# Autodesk Inventor assembly: 276-2156
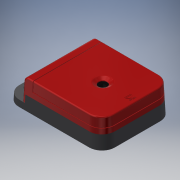
[picture p0: Inventor's stored thumbnail of the model, 180x180]
Saved by Autodesk Inventor 2019.4 (Build 234330000, 330)
## iProperties
Category: Sensors
Company: Autodesk Inc.
Created: 2012-04-02
Part Number: 276-2156
Document SubType Name: Assembly
Designer: Autodesk Inc.
Catalog Web Link: http://www.vexrobotics.com/276-2156.html
Vendor: VEX
Author: Autodesk Inc.
## Documents named in this file (7)
- D:\2019-2020TowerTakeOverCad\ncrCadLib\传感器\Optical Shaft Encoder.iam
- D:\2019-2020TowerTakeOverCad\ncrCadLib\传感器\Reference Parts\Shaft Encoder Bottom.ipt
- D:\2019-2020TowerTakeOverCad\ncrCadLib\传感器\Reference Parts\Optical Shaft Mid.ipt
- D:\2019-2020TowerTakeOverCad\ncrCadLib\传感器\Reference Parts\Shaft Encoder Wheel.ipt
- D:\2019-2020TowerTakeOverCad\ncrCadLib\传感器\Reference Parts\Shaft Encoder Top.ipt
- D:\2019-2020TowerTakeOverCad\ncrCadLib\传感器\Reference Parts\Shaft Encoder Grommet.ipt
- D:\2019-2020TowerTakeOverCad\ncrCadLib\传感器\Reference Parts\ANSI B18.6.3 - 0-80 UNF - 0.1875(5).ipt
## Components (7 placed, 6 different names)
1. Shaft Encoder Bottom:1 — Flush:1, Flush:3, Flush:4, Mate:1, Mate:2, Mate:4, Mate:5, Flush:6, Insert:1, Insert:2
2. Optical Shaft Mid:1 — Flush:1, Flush:3, Flush:4, Flush:5
3. Shaft Encoder Wheel:1 — Mate:1, Mate:2, Mate:3
4. Shaft Encoder Top:1 — Mate:3, Flush:5
5. Shaft Encoder Grommet:1 — Mate:4, Mate:5, Flush:6
6. Cross Recessed Pan Head Machine Screw - Type IA - Inch 0 - 80 - 3/16:1 — Insert:1
7. Cross Recessed Pan Head Machine Screw - Type IA - Inch 0 - 80 - 3/16:2 — Insert:2
## Relationships (12: Flush 5, Mate 5, Insert 2)
- Flush:1: Shaft Encoder Bottom:1 ↔ Optical Shaft Mid:1
- Flush:3: Shaft Encoder Bottom:1 ↔ Optical Shaft Mid:1
- Flush:4: Shaft Encoder Bottom:1 ↔ Optical Shaft Mid:1
- Mate:1: Shaft Encoder Bottom:1 ↔ Shaft Encoder Wheel:1
- Mate:2: Shaft Encoder Bottom:1 ↔ Shaft Encoder Wheel:1
- Mate:3: Shaft Encoder Wheel:1 ↔ Shaft Encoder Top:1
- Flush:5: Optical Shaft Mid:1 ↔ Shaft Encoder Top:1
- Mate:4: Shaft Encoder Bottom:1 ↔ Shaft Encoder Grommet:1
- Mate:5: Shaft Encoder Bottom:1 ↔ Shaft Encoder Grommet:1
- Flush:6: Shaft Encoder Bottom:1 ↔ Shaft Encoder Grommet:1
- Insert:1: Shaft Encoder Bottom:1 ↔ Cross Recessed Pan Head Machine Screw - Type IA - Inch 0 - 80 - 3/16:1
- Insert:2: Shaft Encoder Bottom:1 ↔ Cross Recessed Pan Head Machine Screw - Type IA - Inch 0 - 80 - 3/16:2
